# Autodesk Inventor assembly: 2AM-17-A-6200 - claw arm
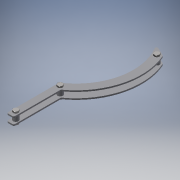
[picture p0: Inventor's stored thumbnail of the model, 180x180]
Saved by Autodesk Inventor 2017 (Build 210142000, 142)
## iProperties
Created: 2017-12-27
Part Number: 2AM-17-A-6200 - claw arm
Document SubType Name: Assembly
Designer: Micah
Author: Micah
## Documents named in this file (5)
- C:\Users\Micah\Desktop\inventor\CADathon-2017\2AM-17-A-0200 - Smokestack Elevator\2AM-17-A-6200 - claw arm.iam
- C:\Users\Micah\Desktop\inventor\CADathon-2017\2AM-17-A-0200 - Smokestack Elevator\2AM-17-P-5201 - claw arm.ipt
- C:\Users\Micah\Desktop\inventor\CADathon-2017\2AM-17-A-0200 - Smokestack Elevator\2AM-17-P-5202 - arm supports.ipt
- C:\Users\Micah\Documents\Inventor\Content Center Files\R2017\en-US\AS 2465(2)\AS 2465 - 1_4 x 1  UNC.ipt
- C:\Users\Micah\Documents\Inventor\Content Center Files\R2017\en-US\AS 2465(3)\AS 2465 - 1_4  UNC(2).ipt
## Components (11 placed, 4 different names)
1. 2AM-17-P-5201 - claw arm:1 — Mate:4, Insert:1, Insert:2, Insert:3
2. 2AM-17-P-5201 - claw arm:2 — Mate:1, Mate:2, Mate:3, Insert:4, Insert:5, Insert:6
3. 2AM-17-P-5202 - arm supports:1 — Mate:1, Mate:4
4. 2AM-17-P-5202 - arm supports:2 — Mate:2
5. 2AM-17-P-5202 - arm supports:3 — Mate:3
6. AS 2465 - Inch 1/4 x 1  UNC:1 — Insert:1
7. AS 2465 - Inch 1/4 x 1  UNC:2 — Insert:2
8. AS 2465 - Inch 1/4 x 1  UNC:3 — Insert:3
9. AS 2465 (Unified hexagon bolts, screws and nuts (UNC and UNF threads) - Inch 1/4  UNC:1 — Insert:4
10. AS 2465 (Unified hexagon bolts, screws and nuts (UNC and UNF threads) - Inch 1/4  UNC:2 — Insert:5
11. AS 2465 (Unified hexagon bolts, screws and nuts (UNC and UNF threads) - Inch 1/4  UNC:3 — Insert:6
## Relationships (10: Insert 6, Mate 4)
- Mate:1: 2AM-17-P-5201 - claw arm:2 ↔ 2AM-17-P-5202 - arm supports:1
- Mate:2: 2AM-17-P-5201 - claw arm:2 ↔ 2AM-17-P-5202 - arm supports:2
- Mate:3: 2AM-17-P-5201 - claw arm:2 ↔ 2AM-17-P-5202 - arm supports:3
- Mate:4: 2AM-17-P-5201 - claw arm:1 ↔ 2AM-17-P-5202 - arm supports:1
- Insert:1: 2AM-17-P-5201 - claw arm:1 ↔ AS 2465 - Inch 1/4 x 1  UNC:1
- Insert:2: 2AM-17-P-5201 - claw arm:1 ↔ AS 2465 - Inch 1/4 x 1  UNC:2
- Insert:3: 2AM-17-P-5201 - claw arm:1 ↔ AS 2465 - Inch 1/4 x 1  UNC:3
- Insert:4: 2AM-17-P-5201 - claw arm:2 ↔ AS 2465 (Unified hexagon bolts, screws and nuts (UNC and UNF threads) - Inch 1/4  UNC:1
- Insert:5: 2AM-17-P-5201 - claw arm:2 ↔ AS 2465 (Unified hexagon bolts, screws and nuts (UNC and UNF threads) - Inch 1/4  UNC:2
- Insert:6: 2AM-17-P-5201 - claw arm:2 ↔ AS 2465 (Unified hexagon bolts, screws and nuts (UNC and UNF threads) - Inch 1/4  UNC:3
